# Autodesk Inventor assembly: Assembly1
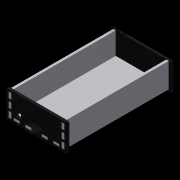
[picture p0: Inventor's stored thumbnail of the model, 180x180]
Saved by Autodesk Inventor 2018 (Build 220112000, 112)
## iProperties
Created: 2018-03-12
Part Number: Assembly1
Document SubType Name: Assembly
Designer: gaine
Author: gaine
## Documents named in this file (5)
- C:\Users\gaine\OneDrive\Documents\Tester Case\Assembly1.iam
- C:\Users\gaine\OneDrive\Documents\Tester Case\Tester Cheek PE.ipt
- C:\Users\gaine\OneDrive\Documents\Tester Case\Tester Cheek NPE.ipt
- C:\Users\gaine\OneDrive\Documents\Tester Case\Front_Back.ipt
- C:\Users\gaine\OneDrive\Documents\Tester Case\Bottom.ipt
## Components (5 placed, 4 different names)
1. Tester Cheek PE:1 — Mate:7, Mate:8, Flush:1, Mate:9, Mate:10, Flush:2, Mate:11, Mate:12, Flush:3, Mate:13, Mate:14, Flush:4
2. Tester Cheek NPE:1 — Mate:1, Mate:2, Mate:3, Mate:4, Mate:5, Mate:6
3. Front_Back:1 — Mate:1, Mate:3, Mate:6
4. Front_Back:2 — Mate:2, Mate:4, Mate:5, Mate:7, Mate:8, Flush:1, Mate:9, Mate:10, Flush:2
5. Bottom:1 — Mate:11, Mate:12, Flush:3, Mate:13, Mate:14, Flush:4
## Relationships (18: Mate 14, Flush 4)
- Mate:1: Tester Cheek NPE:1 ↔ Front_Back:1
- Mate:2: Tester Cheek NPE:1 ↔ Front_Back:2
- Mate:3: Tester Cheek NPE:1 ↔ Front_Back:1
- Mate:4: Tester Cheek NPE:1 ↔ Front_Back:2
- Mate:5: Tester Cheek NPE:1 ↔ Front_Back:2
- Mate:6: Tester Cheek NPE:1 ↔ Front_Back:1
- Mate:7: Tester Cheek PE:1 ↔ Front_Back:2
- Mate:8: Tester Cheek PE:1 ↔ Front_Back:2
- Flush:1: Tester Cheek PE:1 ↔ Front_Back:2
- Mate:9: Tester Cheek PE:1 ↔ Front_Back:2
- Mate:10: Tester Cheek PE:1 ↔ Front_Back:2
- Flush:2: Tester Cheek PE:1 ↔ Front_Back:2
- Mate:11: Tester Cheek PE:1 ↔ Bottom:1
- Mate:12: Tester Cheek PE:1 ↔ Bottom:1
- Flush:3: Tester Cheek PE:1 ↔ Bottom:1
- Mate:13: Tester Cheek PE:1 ↔ Bottom:1
- Mate:14: Tester Cheek PE:1 ↔ Bottom:1
- Flush:4: Tester Cheek PE:1 ↔ Bottom:1
